# Autodesk Inventor assembly: FullAssembly
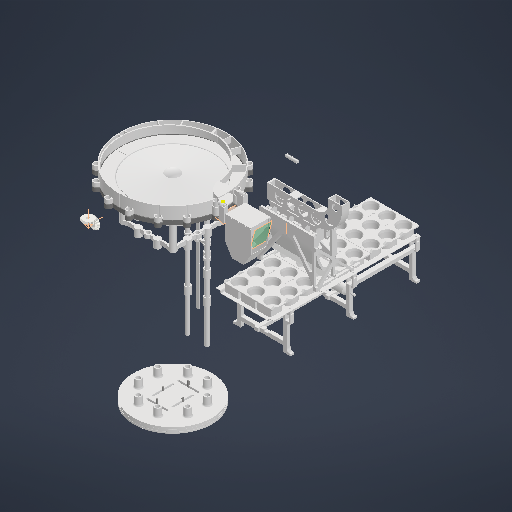
[picture p0: Inventor's stored thumbnail of the model, 512x512]
Saved by Autodesk Inventor 2026.3 (Build 303398000, 398)
## iProperties
Created: 2026-05-08
Part Number: FullAssembly
Document SubType Name: Assembly
Designer: sniel
Author: sniel
## Documents named in this file (5)
- E:\Git\AppliedAutomationProject\CAD\feeder\FullAssembly.iam
- E:\Git\AppliedAutomationProject\CAD\feeder\FeederV3.iam
- E:\Git\AppliedAutomationProject\CAD\feeder\trayFeeder\TrayFeeder.iam
- E:\Git\AppliedAutomationProject\CAD\feeder\table.ipt
- E:\Git\AppliedAutomationProject\CAD\feeder\tableStand.iam
## Components (4 placed, 4 different names)
1. FeederV3:1 [sub-assembly] — Mate:2, Angle:1
2. TrayFeeder:1 [sub-assembly] — Mate:1
3. table:1 — Mate:1
4. tableStand:1 [sub-assembly] — Mate:2, Angle:1
## Relationships (3: Mate 2, Angle 1)
- Mate:1: TrayFeeder:1 ↔ table:1
- Mate:2: FeederV3:1 ↔ tableStand:1
- Angle:1 (0 deg): FeederV3:1 ↔ tableStand:1
